# Autodesk Inventor assembly: top roller
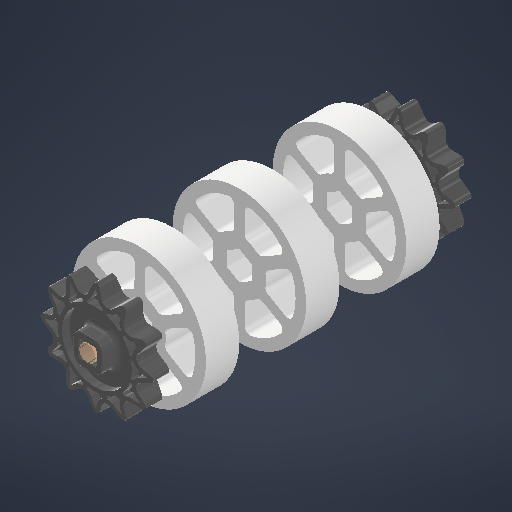
[picture p0: Inventor's stored thumbnail of the model, 512x512]
Saved by Autodesk Inventor 2025.2 (Build 292293000, 293)
## iProperties
Created: 2025-12-04
Part Number: top roller
Document SubType Name: Assembly
Designer: cloudy
Author: cloudy
## Documents named in this file (5)
- C:\Users\cloudy\Documents\GitHub\aura-cad\15\top roller.iam
- C:\Users\cloudy\Documents\GitHub\aura-cad\!lib\Motion\Sprockets\9P Sprocket\9P 12T Sprocket, No Insert.iam
- C:\Users\cloudy\Documents\GitHub\aura-cad\!lib\Motion\Sprockets\9P Sprocket.iam
- C:\Users\cloudy\Documents\GitHub\aura-cad\!lib\Motion\Wheels\Flex Wheels\2.000 Flex Wheel\2.000 30A .500.ipt
- C:\Users\cloudy\Documents\GitHub\aura-cad\!lib\Motion\Wheels\Flex Wheels\2.000 Flex Wheel.ipt
## Components (5 placed, 2 different names)
1. 9P 12T Sprocket, No Insert:1 [sub-assembly]
2. 9P 12T Sprocket, No Insert:2 [sub-assembly]
3. 2.000 30A .500:1
4. 2.000 30A .500:2
5. 2.000 30A .500:3
## Relationships (4: Insert 4)
- [Insert] (6.35 mm): 9P 12T Sprocket, No Insert:1 ↔ 2.000 30A .500:1
- [Insert] (25.4 mm): 2.000 30A .500:1 ↔ 2.000 30A .500:2
- [Insert] (25.4 mm): 2.000 30A .500:2 ↔ 2.000 30A .500:3
- [Insert] (6.35 mm): 9P 12T Sprocket, No Insert:2 ↔ 2.000 30A .500:3
## Named parameters: d0_d1 = 6.35 mm, d1_d2 = 25.4 mm, d2_d3 = 25.4 mm
